# Autodesk Inventor assembly: Carrello
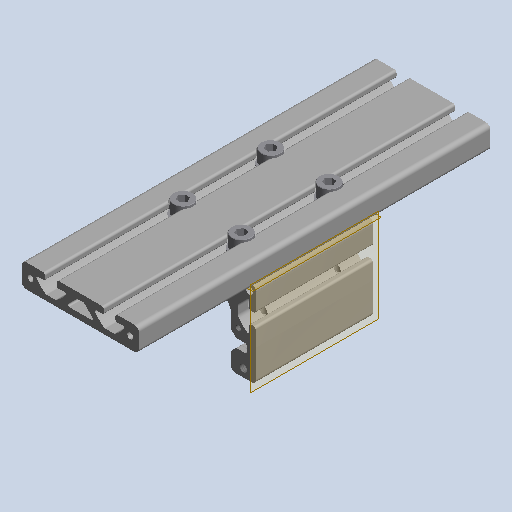
[picture p0: Inventor's stored thumbnail of the model, 512x512]
Saved by Autodesk Inventor 2022 (Build 260153000, 153)
## iProperties
RuleStatus: InUse
Part Number: Carrello
Document SubType Name: Assieme
Designer: matte
Author: matte
## Documents named in this file (4)
- C:\Users\matte\Documents\GitHub\MDM-CyberOrto-CAD\Carrello.iam
- C:\Users\matte\Documents\GitHub\MDM-CyberOrto-CAD\Parker components\08-Linear Application\06-Linear Roller System\01-Roller System 6\30-402.ipt
- C:\Users\matte\Documents\GitHub\MDM-CyberOrto-CAD\Pezzi singoli\Supporto lineare\Piastra.ipt
- C:\Users\matte\Documents\GitHub\MDM-CyberOrto-CAD\Pezzi singoli\Supporto lineare\Giuntura.iam
## Components (7 placed, 4 different names)
1. Piastra:1 — Coincidente:1, Coincidente:2, Coincidente:3, Coincidente:4, Allineato:1, Allineato:2, Coincidente:5, Allineato:3, Coincidente:6, Coincidente:8, Coincidente:9, Coincidente:10
2. Carrello DX — Coincidente:4, Allineato:1, Allineato:2, Allineato:4, Angolo:1, Coincidente:7
3. Carrello SX — Coincidente:5, Allineato:3, Allineato:4
4. Giuntura:1 [sub-assembly] — Coincidente:6, Angolo:1, Coincidente:7, Allineato:5, Allineato:6, Angolo:2
5. Giuntura:2 [sub-assembly] — Coincidente:8, Allineato:5, Allineato:6, Allineato:9
6. Giuntura:3 [sub-assembly] — Coincidente:10
7. Giuntura:4 [sub-assembly] — Coincidente:9, Allineato:9, Angolo:2
## Relationships (21: Mate 10, Flush 9, Angle 2)
- Coincidente:1 [Mate]: Piastra:1
- Coincidente:2 [Mate]: Piastra:1
- Coincidente:3 [Mate]: Piastra:1
- Coincidente:4 [Mate]: Piastra:1 ↔ Carrello DX
- Allineato:1 [Flush]: Piastra:1 ↔ Carrello DX
- Allineato:2 [Flush] (80 mm): Piastra:1 ↔ Carrello DX
- Coincidente:5 [Mate]: Piastra:1 ↔ Carrello SX
- Allineato:3 [Flush]: Piastra:1 ↔ Carrello SX
- Allineato:4 [Flush]: Carrello DX ↔ Carrello SX
- Coincidente:6 [Mate]: Piastra:1 ↔ Giuntura:1
- Angolo:1 [Angle] (0 deg): Carrello DX ↔ Giuntura:1
- Coincidente:7 [Mate]: Carrello DX ↔ Giuntura:1
- Coincidente:8 [Mate]: Piastra:1 ↔ Giuntura:2
- Allineato:5 [Flush]: Giuntura:1 ↔ Giuntura:2
- Allineato:6 [Flush]: Giuntura:1 ↔ Giuntura:2
- [Flush]: Giuntura:3 ↔ Giuntura:4
- [Flush]: Giuntura:3 ↔ Giuntura:4
- Coincidente:9 [Mate]: Piastra:1 ↔ Giuntura:4
- Allineato:9 [Flush]: Giuntura:2 ↔ Giuntura:4
- Angolo:2 [Angle] (180 deg): Giuntura:1 ↔ Giuntura:4
- Coincidente:10 [Mate]: Piastra:1 ↔ Giuntura:3
## Named parameters: L_piatto = 240 mm, d38_d36 = 0 mm, d39_d37 = 0 mm
